# Autodesk Inventor assembly: 装配-刮肉轮
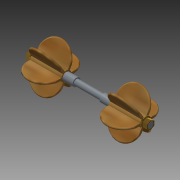
[picture p0: Inventor's stored thumbnail of the model, 180x180]
Saved by Autodesk Inventor 2015 (Build 190159000, 159)
## iProperties
Created: 2017-05-24
Part Number: 装配-刮肉轮
Document SubType Name: Assembly
Designer: Administrator
Author: Administrator
## Documents named in this file (4)
- C:\Users\Administrator\Desktop\毕设改\装配-刮肉轮.iam
- C:\Users\Administrator\Desktop\毕设改\刮肉轮.ipt
- C:\Users\Administrator\Desktop\毕设改\刮肉轮固定螺丝.ipt
- C:\Users\Administrator\Desktop\毕设改\刮肉轮轴.ipt
## Components (5 placed, 3 different names)
1. 刮肉轮:1 — 插入:1, 插入:2, 表面齐平:1
2. 刮肉轮固定螺丝:1 — 插入:2
3. 刮肉轮轴:1 — 插入:1, 插入:4
4. 刮肉轮:2 — 插入:4, 表面齐平:1
5. 刮肉轮固定螺丝:2
## Relationships (5: Insert 4, Flush 1)
- 插入:1 [Insert]: 刮肉轮:1 ↔ 刮肉轮轴:1
- 插入:2 [Insert]: 刮肉轮:1 ↔ 刮肉轮固定螺丝:1
- [Insert]: 刮肉轮:2 ↔ 刮肉轮固定螺丝:2
- 插入:4 [Insert]: 刮肉轮轴:1 ↔ 刮肉轮:2
- 表面齐平:1 [Flush]: 刮肉轮:1 ↔ 刮肉轮:2
## Named parameters: d2_d1 = 0 mm
